# Autodesk Inventor assembly: Exploration
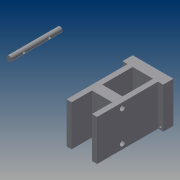
[picture p0: Inventor's stored thumbnail of the model, 180x180]
Saved by Autodesk Inventor 2019 (Build 230136000, 136)
## iProperties
Created: 2020-02-17
Part Number: Exploration
Document SubType Name: Assembly
Designer: Goutham
Author: Goutham
## Documents named in this file (4)
- C:\Users\Goutham\Documents\S.Mech\Exploration.iam
- C:\Users\Goutham\Documents\S.Mech\Expo.ipt
- C:\Users\Goutham\Documents\S.Mech\Expo_2.ipt
- C:\Users\Goutham\Documents\S.Mech\Expo_1.ipt
## Components (3 placed, 3 different names)
1. Expo:1 — Mate:1, Mate:2, Mate:3
2. Expo_2:1 — Mate:1, Mate:2, Mate:3
3. Expo_1:1
## Relationships (3: Mate 3)
- Mate:1: Expo:1 ↔ Expo_2:1
- Mate:2: Expo:1 ↔ Expo_2:1
- Mate:3: Expo:1 ↔ Expo_2:1
